# Autodesk Inventor assembly: V4 Assembly
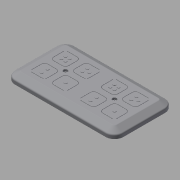
[picture p0: Inventor's stored thumbnail of the model, 180x180]
Saved by Autodesk Inventor 2018 (Build 220112000, 112)
## iProperties
Created: 2020-01-10
Part Number: V4 Assembly
Document SubType Name: Assembly
Designer: user
Author: user
## Documents named in this file (3)
- C:\Users\user\Google Drive\Projects\3d\4 Projects\Smart switch\V4 Assembly.iam
- C:\Users\user\Google Drive\Projects\3d\4 Projects\Smart switch\V4 dual in wall.ipt
- C:\Users\user\Google Drive\Projects\3d\4 Projects\Smart switch\V4 dual.ipt
## Components (2 placed, 2 different names)
1. V4 dual in wall:1 — Flush:1, Mate:1, Mate:2
2. V4 dual:1 — Flush:1, Mate:1, Mate:2
## Relationships (3: Mate 2, Flush 1)
- Flush:1: V4 dual in wall:1 ↔ V4 dual:1
- Mate:1: V4 dual in wall:1 ↔ V4 dual:1
- Mate:2: V4 dual in wall:1 ↔ V4 dual:1
